# Autodesk Inventor assembly: CH-2-01-Chassis Assembly
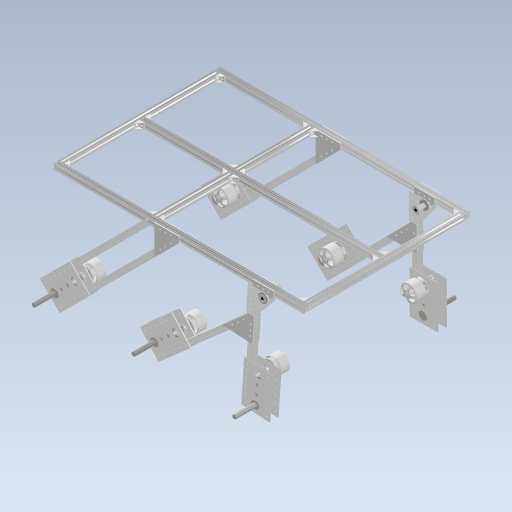
[picture p0: Inventor's stored thumbnail of the model, 512x512]
Saved by Autodesk Inventor 2023 (Build 270158000, 158)
## iProperties
Created: 2023-02-17
Part Number: CH-2-01-Chassis Assembly
Document SubType Name: Assembly
Designer: Dave
Author: Dave
## Documents named in this file (8)
- C:\Users\Dave\Documents\GitHub\BehrendURCMechanical\CAD\Chassis\CH-2-01-Chassis Assembly.iam
- C:\Users\Dave\Documents\GitHub\BehrendURCMechanical\CAD\Chassis\GearBox\Final Gears and Assemblies\FrontGearboxAssembly.iam
- C:\Users\Dave\Documents\GitHub\BehrendURCMechanical\CAD\Chassis\GearBox\Final Gears and Assemblies\RearGearboxAssembly.iam
- C:\Users\Dave\Documents\GitHub\BehrendURCMechanical\CAD\Chassis\CH-1-01-BearingBracket.ipt
- C:\Users\Dave\Documents\GitHub\BehrendURCMechanical\CAD\Chassis\GearBox\Final Gears and Assemblies\FrontGearboxAssembly_MIR.iam
- C:\Users\Dave\Documents\GitHub\BehrendURCMechanical\CAD\Chassis\GearBox\Final Gears and Assemblies\RearGearboxAssembly_MIR.iam
- C:\Users\Dave\Documents\GitHub\BehrendURCMechanical\CAD\Chassis\CH-1-01-BearingBracket_MIR.ipt
- C:\Users\Dave\Documents\GitHub\BehrendURCMechanical\CAD\Chassis\Ch-0-02-ChassisFrame.iam
## Components (7 placed, 7 different names)
1. FrontGearboxAssembly:1 [sub-assembly] — Mate:5, Mate:15
2. RearGearboxAssembly:1 [sub-assembly] — Tangent:1, Flush:8, Mate:10, Flush:12
3. Ch-0-02-ChassisFrame:1 [sub-assembly] — Mate:8, Mate:9, Mate:10, Mate:11, Mate:12, Mate:13, Mate:14, Mate:15, Mate:16, Flush:11, Flush:12, Tangent:3, Tangent:4
4. CH-1-01-BearingBracket:1 — Mate:5, Flush:10, Mate:12, Mate:13
5. FrontGearboxAssembly_MIR:1 [sub-assembly] — Mate:7, Mate:14, Tangent:4
6. RearGearboxAssembly_MIR:1 [sub-assembly] — Tangent:2, Flush:8, Mate:9, Mate:16, Flush:11, Tangent:3
7. CH-1-01-BearingBracket_MIR:1 — Mate:7, Flush:10, Mate:8, Mate:11
## Relationships (22: Mate 11, Flush 7, Tangent 4)
- [Flush]: Ch-0-02-ChassisFrame:1
- [Flush]: Ch-0-02-ChassisFrame:1
- [Flush]: Ch-0-02-ChassisFrame:1
- Tangent:1: RearGearboxAssembly:1
- Mate:5: FrontGearboxAssembly:1 ↔ CH-1-01-BearingBracket:1
- Tangent:2: RearGearboxAssembly_MIR:1
- Mate:7: FrontGearboxAssembly_MIR:1 ↔ CH-1-01-BearingBracket_MIR:1
- Flush:8: RearGearboxAssembly:1 ↔ RearGearboxAssembly_MIR:1
- Flush:10: CH-1-01-BearingBracket:1 ↔ CH-1-01-BearingBracket_MIR:1
- Mate:8: Ch-0-02-ChassisFrame:1 ↔ CH-1-01-BearingBracket_MIR:1
- Mate:9: Ch-0-02-ChassisFrame:1 ↔ RearGearboxAssembly_MIR:1
- Mate:10: RearGearboxAssembly:1 ↔ Ch-0-02-ChassisFrame:1
- Mate:11: Ch-0-02-ChassisFrame:1 ↔ CH-1-01-BearingBracket_MIR:1
- Mate:12: Ch-0-02-ChassisFrame:1 ↔ CH-1-01-BearingBracket:1
- Mate:13: Ch-0-02-ChassisFrame:1 ↔ CH-1-01-BearingBracket:1
- Mate:14: Ch-0-02-ChassisFrame:1 ↔ FrontGearboxAssembly_MIR:1
- Mate:15: FrontGearboxAssembly:1 ↔ Ch-0-02-ChassisFrame:1
- Mate:16: Ch-0-02-ChassisFrame:1 ↔ RearGearboxAssembly_MIR:1
- Flush:11: Ch-0-02-ChassisFrame:1 ↔ RearGearboxAssembly_MIR:1
- Flush:12: RearGearboxAssembly:1 ↔ Ch-0-02-ChassisFrame:1
- Tangent:3: Ch-0-02-ChassisFrame:1 ↔ RearGearboxAssembly_MIR:1
- Tangent:4 (127 mm): Ch-0-02-ChassisFrame:1 ↔ FrontGearboxAssembly_MIR:1
